# Autodesk Inventor assembly: ExpansionCard4
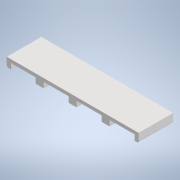
[picture p0: Inventor's stored thumbnail of the model, 180x180]
Saved by Autodesk Inventor 2022 (Build 260153000, 153)
## iProperties
Created: 2021-11-01
Part Number: ExpansionCard4
Document SubType Name: Assembly
Designer: Josh
Author: Josh
## Documents named in this file (2)
- C:\Users\Josh\Documents\ExpansionCard4.iam
- C:\Users\Josh\Documents\ExpansionCard1.ipt
## Components (4 placed, 1 different names)
1. ExpansionCard1:1 — Rigid:1, Rigid:2
2. ExpansionCard1:2 — Rigid:1
3. ExpansionCard1:3 — Rigid:3
4. ExpansionCard1:4 — Rigid:2, Rigid:3
## Relationships (3: WeldJoint 3)
- Rigid:1 [WeldJoint]: ExpansionCard1:1 ↔ ExpansionCard1:2
- Rigid:2 [WeldJoint]: ExpansionCard1:1 ↔ ExpansionCard1:4
- Rigid:3 [WeldJoint]: ExpansionCard1:3 ↔ ExpansionCard1:4
